# Autodesk Inventor assembly: cylinder_aq232x500
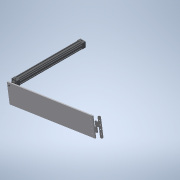
[picture p0: Inventor's stored thumbnail of the model, 180x180]
Saved by Autodesk Inventor 2022 (Build 260153000, 153)
## iProperties
Created: 2022-10-26
Part Number: cylinder_aq232x500
Checked By: TraceParts S.A.
Catalog Web Link: www.traceparts.com
Document SubType Name: Assembly
Designer: TraceParts
Company: TraceParts S.A.
REFERENCE: AQ232X500
SUPPLIER: CHANTO AIR HYDRAULICS CO., LTD.
DESIGN: AQ2 ISO cylinder ISO6431,VDMA24562 AQ232X500
TraceParts.PartNumber: 33-28012019-057283
TraceParts.PartTitle: AQ2 ISO cylinder ISO6431,VDMA24562 AQ232X500
TraceParts.InstanceId: 33-28012019-0572839T75CBMCI0X913BHFYCWRSKYX
TRACEPARTS: TRACEPARTS
TraceParts.PartLanguage: en
TraceParts.PartVersion: 1.1.7
Author: TraceParts
## Documents named in this file (6)
- C:\Users\USUARIO\Documents\Academico\2023-I\APM\Proyecto\Gemelo Digital\Empaquetado\Actuador\cylinder_aq232x500.iam
- C:\Users\USUARIO\Documents\Academico\2023-I\APM\Proyecto\Gemelo Digital\Empaquetado\Actuador\cylinder_aq232x500_01.ipt
- C:\Users\USUARIO\Documents\Academico\2023-I\APM\Proyecto\Gemelo Digital\Empaquetado\Actuador\cylinder_aq232x500_02.ipt
- C:\Users\USUARIO\Documents\Academico\2023-I\APM\Proyecto\Gemelo Digital\Empaquetado\Actuador\cylinder_aq232x500_03.ipt
- C:\Users\USUARIO\Documents\Academico\2023-I\APM\Proyecto\Gemelo Digital\Empaquetado\Actuador\Ensamblaje-Bisagra_inv.iam
- C:\Users\USUARIO\Documents\Academico\2023-I\APM\Proyecto\Gemelo Digital\Empaquetado\Actuador\Tabla_movimiento.ipt
## Components (5 placed, 5 different names)
1. cylinder_aq232x500_01:1
2. cylinder_aq232x500_02:1 — Coincidencia:1
3. cylinder_aq232x500_03:1 — Coincidencia:2
4. Ensamblaje-Bisagra_inv:1 [sub-assembly] — Coincidencia:3, Coincidencia:4, Coincidencia:5
5. Tabla_movimiento:1 — Coincidencia:1, Coincidencia:2, Coincidencia:3, Coincidencia:4, Coincidencia:5
## Relationships (5: Mate 5)
- Coincidencia:1 [Mate]: cylinder_aq232x500_02:1 ↔ Tabla_movimiento:1
- Coincidencia:2 [Mate]: cylinder_aq232x500_03:1 ↔ Tabla_movimiento:1
- Coincidencia:3 [Mate]: Ensamblaje-Bisagra_inv:1 ↔ Tabla_movimiento:1
- Coincidencia:4 [Mate]: Ensamblaje-Bisagra_inv:1 ↔ Tabla_movimiento:1
- Coincidencia:5 [Mate]: Ensamblaje-Bisagra_inv:1 ↔ Tabla_movimiento:1
